# Autodesk Inventor assembly: Joes_Robot
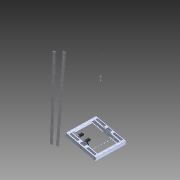
[picture p0: Inventor's stored thumbnail of the model, 180x180]
Saved by Autodesk Inventor 2015 SP1 (Build 190203100, 203)
## iProperties
Created: 2015-01-23
Part Number: Joes_Robot
Document SubType Name: Assembly
Designer: 55221
Author: 55221
## Documents named in this file (18)
- Z:\RoboEaglesCAD\Joes_Robot.iam
- Z:\RoboEaglesCAD\wheelBase\Outside Sheet Square.ipt
- Z:\RoboEaglesCAD\wheelBase\2x3 Hole Bracket.ipt
- Z:\RoboEaglesCAD\wheelBase\Inside Sheet Square.ipt
- Z:\RoboEaglesCAD\wheelBase\End Sheet Square.ipt
- Z:\RoboEaglesCAD\Motion\GuidanceShaft.ipt
- Z:\RoboEaglesCAD\Motion\Roller.ipt
- Z:\RoboEaglesCAD\wheelBase\churroLong.ipt
- Z:\RoboEaglesCAD\wheelBase\TM Housing.ipt
- Z:\RoboEaglesCAD\wheelBase\TB Output Shaft Hex L-Base 2.ipt
- Z:\RoboEaglesCAD\wheelBase\GBBearing.ipt
- Z:\RoboEaglesCAD\wheelBase\Hex Bearing.ipt
- Z:\RoboEaglesCAD\wheelBase\CIM Motor SW.ipt
- Z:\RoboEaglesCAD\Bolt&nut.iam
- Z:\RoboEaglesCAD\wheelBase\gearBoxSimple\simpleGBHousing.ipt
- Z:\RoboEaglesCAD\wheelBase\gearBoxSimple\simpleGBMount.ipt
- Z:\RoboEaglesCAD\wheelBase\gearBoxSimple\simpleGBStopBlockSmallCylindrical.ipt
- Z:\RoboEaglesCAD\wheelBase\gearBoxSimple\simpleGBStopBlockLargeHex.ipt
## Components (30 placed, 17 different names)
1. Outside Sheet Square:1 — Mate:1, Mate:2, Mate:3, Mate:7, Mate:9, Mate:10, Mate:12, Mate:13, Mate:14, Mate:33, Mate:34, Mate:88, Mate:89
2. 2x3 Hole Bracket:1 — Mate:7, Mate:8, Mate:9, Mate:10, Mate:11
3. 2x3 Hole Bracket:2 — Mate:1, Mate:2, Mate:3, Mate:4, Mate:5, Mate:6
4. Inside Sheet Square:1 — Mate:4, Mate:5, Mate:6, Mate:8, Mate:11, Mate:15, Mate:16, Mate:36, Mate:37, Mate:81, Mate:82, Mate:83, Mate:100, Mate:101, Mate:113, Mate:114
5. End Sheet Square:1 — Mate:12, Mate:13, Mate:14, Mate:15, Mate:16, Mate:17, Mate:18, Mate:19, Mate:46
6. Inside Sheet Square:2 — Mate:23, Mate:35, Mate:42, Mate:43, Mate:44, Mate:45, Mate:46, Mate:47, Mate:50, Mate:51
7. Outside Sheet Square:2 — Mate:17, Mate:18, Mate:19, Mate:20, Mate:21, Mate:22, Mate:28, Mate:29, Mate:30, Mate:40, Mate:41
8. End Sheet Square:2 — Mate:33, Mate:34, Mate:35, Mate:36, Mate:37, Mate:40, Mate:41, Mate:47, Angle:3
9. 2x3 Hole Bracket:3 — Mate:20, Mate:21, Mate:22, Mate:23, Mate:44, Mate:45
10. 2x3 Hole Bracket:4 — Mate:28, Mate:29, Mate:30, Mate:42, Mate:43
11. GuidanceShaft:1
12. GuidanceShaft:2
13. Roller:1
14. churroLong:2 — Mate:50, Mate:51
15. TM Housing:1 — Mate:81, Mate:82, Mate:83, Mate:84, Mate:85, Mate:91, Mate:93, Mate:94, Mate:95, Mate:96, Mate:97, Mate:98, Mate:99
16. GBBearing:2
17. GBBearing:3 — Mate:84, Mate:85, Mate:86, Mate:87
18. TB Output Shaft Hex L-Base 2:2 — Mate:86, Mate:87, Angle:2
19. Hex Bearing:2 — Mate:88, Mate:89, Angle:2
20. CIM Motor SW:3 — Mate:111, Mate:112
21. CIM Motor SW:4 — Mate:91, Mate:93
22. Bolt&nut:1 [sub-assembly] — Mate:94, Mate:95
23. Bolt&nut:2 [sub-assembly] — Mate:98, Mate:100
24. Bolt&nut:3 [sub-assembly] — Mate:99, Mate:101
25. Bolt&nut:4 [sub-assembly] — Mate:96, Mate:97
26. simpleGBHousing:1 — Mate:102, Mate:103, Mate:104, Mate:105, Mate:106, Mate:109, Mate:110, Mate:111, Mate:112, Angle:3
27. simpleGBMount:1 — Mate:102, Mate:103, Mate:104
28. TB Output Shaft Hex L-Base 2:3 — Mate:107, Mate:108
29. simpleGBStopBlockSmallCylindrical:1 — Mate:105, Mate:106, Mate:107, Mate:108
30. simpleGBStopBlockLargeHex:1 — Mate:109, Mate:110, Mate:113, Mate:114
## Relationships (75: Mate 73, Angle 2)
- Mate:1: Outside Sheet Square:1 ↔ 2x3 Hole Bracket:2
- Mate:2: Outside Sheet Square:1 ↔ 2x3 Hole Bracket:2
- Mate:3: Outside Sheet Square:1 ↔ 2x3 Hole Bracket:2
- Mate:4: 2x3 Hole Bracket:2 ↔ Inside Sheet Square:1
- Mate:5: 2x3 Hole Bracket:2 ↔ Inside Sheet Square:1
- Mate:6: 2x3 Hole Bracket:2 ↔ Inside Sheet Square:1
- Mate:7: Outside Sheet Square:1 ↔ 2x3 Hole Bracket:1
- Mate:8: 2x3 Hole Bracket:1 ↔ Inside Sheet Square:1
- Mate:9: Outside Sheet Square:1 ↔ 2x3 Hole Bracket:1
- Mate:10: Outside Sheet Square:1 ↔ 2x3 Hole Bracket:1
- Mate:11: 2x3 Hole Bracket:1 ↔ Inside Sheet Square:1
- Mate:12: Outside Sheet Square:1 ↔ End Sheet Square:1
- Mate:13: Outside Sheet Square:1 ↔ End Sheet Square:1
- Mate:14: Outside Sheet Square:1 ↔ End Sheet Square:1
- Mate:15: Inside Sheet Square:1 ↔ End Sheet Square:1
- Mate:16: Inside Sheet Square:1 ↔ End Sheet Square:1
- Mate:17: End Sheet Square:1 ↔ Outside Sheet Square:2
- Mate:18: End Sheet Square:1 ↔ Outside Sheet Square:2
- Mate:19: End Sheet Square:1 ↔ Outside Sheet Square:2
- Mate:20: Outside Sheet Square:2 ↔ 2x3 Hole Bracket:3
- Mate:21: Outside Sheet Square:2 ↔ 2x3 Hole Bracket:3
- Mate:22: Outside Sheet Square:2 ↔ 2x3 Hole Bracket:3
- Mate:23: Inside Sheet Square:2 ↔ 2x3 Hole Bracket:3
- Mate:28: Outside Sheet Square:2 ↔ 2x3 Hole Bracket:4
- Mate:29: Outside Sheet Square:2 ↔ 2x3 Hole Bracket:4
- Mate:30: Outside Sheet Square:2 ↔ 2x3 Hole Bracket:4
- Mate:33: Outside Sheet Square:1 ↔ End Sheet Square:2
- Mate:34: Outside Sheet Square:1 ↔ End Sheet Square:2
- Mate:35: Inside Sheet Square:2 ↔ End Sheet Square:2
- Mate:36: Inside Sheet Square:1 ↔ End Sheet Square:2
- Mate:37: Inside Sheet Square:1 ↔ End Sheet Square:2
- Mate:40: Outside Sheet Square:2 ↔ End Sheet Square:2
- Mate:41: Outside Sheet Square:2 ↔ End Sheet Square:2
- Mate:42: Inside Sheet Square:2 ↔ 2x3 Hole Bracket:4
- Mate:43: Inside Sheet Square:2 ↔ 2x3 Hole Bracket:4
- Mate:44: Inside Sheet Square:2 ↔ 2x3 Hole Bracket:3
- Mate:45: Inside Sheet Square:2 ↔ 2x3 Hole Bracket:3
- Mate:46: End Sheet Square:1 ↔ Inside Sheet Square:2
- Mate:47: Inside Sheet Square:2 ↔ End Sheet Square:2
- Mate:50: Inside Sheet Square:2 ↔ churroLong:2
- Mate:51: Inside Sheet Square:2 ↔ churroLong:2
- Mate:81: Inside Sheet Square:1 ↔ TM Housing:1
- Mate:82: Inside Sheet Square:1 ↔ TM Housing:1
- Mate:83: Inside Sheet Square:1 ↔ TM Housing:1
- Mate:84: TM Housing:1 ↔ GBBearing:3
- Mate:85: TM Housing:1 ↔ GBBearing:3
- Mate:86: GBBearing:3 ↔ TB Output Shaft Hex L-Base 2:2
- Mate:87: GBBearing:3 ↔ TB Output Shaft Hex L-Base 2:2
- Mate:88: Outside Sheet Square:1 ↔ Hex Bearing:2
- Mate:89: Outside Sheet Square:1 ↔ Hex Bearing:2
- Angle:2 (0 deg): TB Output Shaft Hex L-Base 2:2 ↔ Hex Bearing:2
- Mate:91: TM Housing:1 ↔ CIM Motor SW:4
- Mate:93: TM Housing:1 ↔ CIM Motor SW:4
- Mate:94: TM Housing:1 ↔ Bolt&nut:1
- Mate:95: TM Housing:1 ↔ Bolt&nut:1
- Mate:96: TM Housing:1 ↔ Bolt&nut:4
- Mate:97: TM Housing:1 ↔ Bolt&nut:4
- Mate:98: TM Housing:1 ↔ Bolt&nut:2
- Mate:99: TM Housing:1 ↔ Bolt&nut:3
- Mate:100: Inside Sheet Square:1 ↔ Bolt&nut:2
- Mate:101: Inside Sheet Square:1 ↔ Bolt&nut:3
- Mate:102: simpleGBHousing:1 ↔ simpleGBMount:1
- Mate:103: simpleGBHousing:1 ↔ simpleGBMount:1
- Mate:104: simpleGBHousing:1 ↔ simpleGBMount:1
- Mate:105: simpleGBHousing:1 ↔ simpleGBStopBlockSmallCylindrical:1
- Mate:106: simpleGBHousing:1 ↔ simpleGBStopBlockSmallCylindrical:1
- Mate:107: TB Output Shaft Hex L-Base 2:3 ↔ simpleGBStopBlockSmallCylindrical:1
- Mate:108: TB Output Shaft Hex L-Base 2:3 ↔ simpleGBStopBlockSmallCylindrical:1
- Mate:109: simpleGBHousing:1 ↔ simpleGBStopBlockLargeHex:1
- Mate:110: simpleGBHousing:1 ↔ simpleGBStopBlockLargeHex:1
- Mate:111: CIM Motor SW:3 ↔ simpleGBHousing:1
- Mate:112: CIM Motor SW:3 ↔ simpleGBHousing:1
- Mate:113: Inside Sheet Square:1 ↔ simpleGBStopBlockLargeHex:1
- Mate:114: Inside Sheet Square:1 ↔ simpleGBStopBlockLargeHex:1
- Angle:3 (0 deg): End Sheet Square:2 ↔ simpleGBHousing:1
